# Autodesk Inventor assembly: j1 assmble
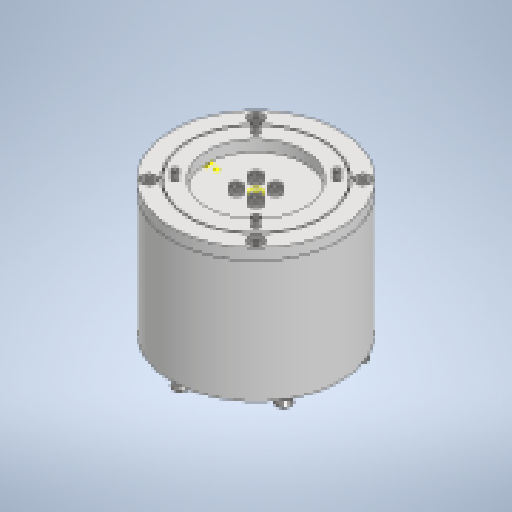
[picture p0: Inventor's stored thumbnail of the model, 512x512]
Saved by Autodesk Inventor 2025 (Build 290162000, 162)
## iProperties
Created: 2025-07-11
Part Number: j1 assmble
Document SubType Name: Assembly
Designer: gavin
Author: gavin
## Documents named in this file (12)
- D:\Inventor\robot armT 2\j1 assmble.iam
- D:\Inventor\robot armT 2\arm bearing.ipt
- D:\Inventor\robot armT 2\nema23_57HS56\nema23_57HS56.ipt
- D:\Inventor\robot armT 2\xl28 driven.ipt
- D:\Inventor\robot armT 2\j1 moving plate.ipt
- D:\Inventor\robot armT 2\j1 57 mount.ipt
- D:\Inventor\robot armT 2\optic endstop module.ipt
- D:\Inventor\robot armT 2\DIN 7991 - M5x12.ipt
- D:\Inventor\robot armT 2\CNS 4557 - M5 x 0.8 x 10.ipt
- D:\Inventor\robot armT 2\DIN 7991 - M5x20.ipt
- D:\Inventor\robot armT 2\j1 endstop block v2.ipt
- D:\Inventor\robot armT 2\BS 4168 - M5 x 16(7).ipt
## Components (29 placed, 11 different names)
1. arm bearing:1
2. nema23_57HS56:1
3. xl28 driven:1
4. j1 moving plate:1 — 齊平:4
5. j1 57 mount:1 — 旋轉:13, 旋轉:14, 旋轉:15, 旋轉:16
6. optic endstop module:1
7. DIN 7991 - M5x12:1
8. DIN 7991 - M5x12:2
9. DIN 7991 - M5x12:3
10. DIN 7991 - M5x12:4
11. DIN 7991 - M5x12:5
12. DIN 7991 - M5x12:6
13. DIN 7991 - M5x12:7
14. DIN 7991 - M5x12:8
15. DIN 7991 - M5x12:9
16. DIN 7991 - M5x12:10
17. CNS 4557 - M5 x 0.8 x 10:1
18. CNS 4557 - M5 x 0.8 x 10:2
19. CNS 4557 - M5 x 0.8 x 10:3
20. CNS 4557 - M5 x 0.8 x 10:4
21. DIN 7991 - M5x20:1
22. DIN 7991 - M5x20:2
23. DIN 7991 - M5x20:3
24. DIN 7991 - M5x20:4
25. j1 endstop block v2:1 — 齊平:4
26. BS 4168 - M5 x 16(7):1 — 旋轉:13
27. BS 4168 - M5 x 16(7):2 — 旋轉:14
28. BS 4168 - M5 x 16(7):3 — 旋轉:16
29. BS 4168 - M5 x 16(7):4 — 旋轉:15
## Relationships (34: RevoluteJoint 16, Mate 14, Flush 4)
- [Mate]: arm bearing:1 ↔ j1 moving plate:1
- [Mate]: arm bearing:1 ↔ j1 moving plate:1
- [Mate]: arm bearing:1 ↔ j1 moving plate:1
- [Mate]: xl28 driven:1 ↔ j1 moving plate:1
- [Mate]: xl28 driven:1 ↔ j1 moving plate:1
- [Mate]: xl28 driven:1 ↔ j1 moving plate:1
- [Mate]: nema23_57HS56:1 ↔ xl28 driven:1
- [Mate]: nema23_57HS56:1 ↔ xl28 driven:1
- [Flush]: nema23_57HS56:1 ↔ j1 57 mount:1
- [Flush]: nema23_57HS56:1 ↔ j1 57 mount:1
- [Flush]: nema23_57HS56:1 ↔ j1 57 mount:1
- [Mate]: nema23_57HS56:1 ↔ j1 57 mount:1
- [Mate]: arm bearing:1 ↔ j1 57 mount:1
- [Mate]: arm bearing:1 ↔ j1 57 mount:1
- [Mate]: j1 57 mount:1 ↔ optic endstop module:1
- [Mate]: j1 57 mount:1 ↔ optic endstop module:1
- [Mate]: j1 57 mount:1 ↔ optic endstop module:1
- [RevoluteJoint]: arm bearing:1 ↔ DIN 7991 - M5x12:1
- [RevoluteJoint]: arm bearing:1 ↔ DIN 7991 - M5x12:6
- [RevoluteJoint]: arm bearing:1 ↔ DIN 7991 - M5x12:5
- [RevoluteJoint]: arm bearing:1 ↔ DIN 7991 - M5x12:2
- [RevoluteJoint]: j1 moving plate:1 ↔ CNS 4557 - M5 x 0.8 x 10:1
- [RevoluteJoint]: j1 moving plate:1 ↔ CNS 4557 - M5 x 0.8 x 10:2
- [RevoluteJoint]: j1 moving plate:1 ↔ CNS 4557 - M5 x 0.8 x 10:3
- [RevoluteJoint]: j1 moving plate:1 ↔ CNS 4557 - M5 x 0.8 x 10:4
- [RevoluteJoint]: j1 moving plate:1 ↔ DIN 7991 - M5x20:1
- [RevoluteJoint]: j1 moving plate:1 ↔ DIN 7991 - M5x20:2
- [RevoluteJoint]: j1 moving plate:1 ↔ DIN 7991 - M5x20:3
- [RevoluteJoint]: j1 moving plate:1 ↔ DIN 7991 - M5x20:4
- 齊平:4 [Flush]: j1 moving plate:1 ↔ j1 endstop block v2:1
- 旋轉:13 [RevoluteJoint]: j1 57 mount:1 ↔ BS 4168 - M5 x 16(7):1
- 旋轉:14 [RevoluteJoint]: j1 57 mount:1 ↔ BS 4168 - M5 x 16(7):2
- 旋轉:15 [RevoluteJoint]: j1 57 mount:1 ↔ BS 4168 - M5 x 16(7):4
- 旋轉:16 [RevoluteJoint]: j1 57 mount:1 ↔ BS 4168 - M5 x 16(7):3
## Named parameters: d34_d40 = 0 mm, d35_d41 = 0 mm
